# Autodesk Inventor assembly: сервомотор
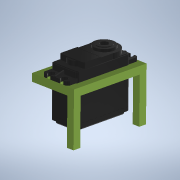
[picture p0: Inventor's stored thumbnail of the model, 180x180]
Saved by Autodesk Inventor 2021.1 (Build 251245010, 245A)
## iProperties
Created: 2022-12-17
Part Number: сервомотор
Document SubType Name: Assembly
Designer: zmoze
Author: zmoze
## Documents named in this file (3)
- C:\Users\zmoze\OneDrive\Рабочий стол\GrabCAD\Smile_2022-2023\сервомотор.iam
- C:\Users\zmoze\OneDrive\Рабочий стол\GrabCAD\Smile_2022-2023\серва_HS485-HB.ipt
- C:\Users\zmoze\OneDrive\Рабочий стол\GrabCAD\Smile_2022-2023\держатель_сервы.ipt
## Components (2 placed, 2 different names)
1. серва_HS485-HB:1 — Совмещение:2, Заподлицо:1, Совмещение:3
2. держатель_сервы:1 — Совмещение:2, Заподлицо:1, Совмещение:3
## Relationships (3: Mate 2, Flush 1)
- Совмещение:2 [Mate]: серва_HS485-HB:1 ↔ держатель_сервы:1
- Заподлицо:1 [Flush] (-0.51 mm): серва_HS485-HB:1 ↔ держатель_сервы:1
- Совмещение:3 [Mate]: серва_HS485-HB:1 ↔ держатель_сервы:1
